# Autodesk Inventor assembly: Assembly_components
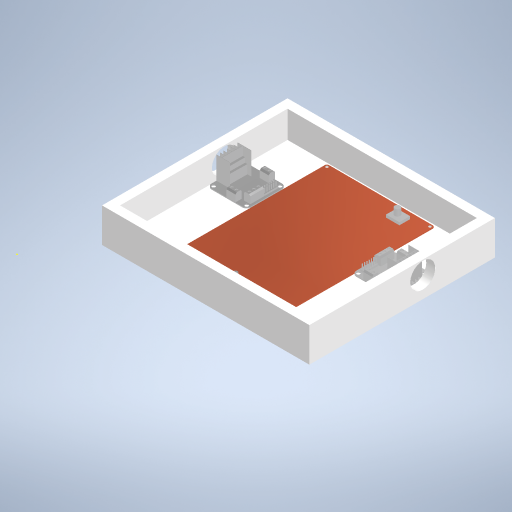
[picture p0: Inventor's stored thumbnail of the model, 512x512]
Saved by Autodesk Inventor 2023 (Build 270158000, 158)
## iProperties
Created: 2023-03-21
Part Number: Assembly_components
Document SubType Name: Assembly
Designer: 55119
Author: 55119
## Documents named in this file (5)
- C:\Users\55119\Documents\GitHub\tectonics\src\3d_models\Case\Assembly_components.iam
- C:\Users\55119\Documents\GitHub\tectonics\src\3d_models\Case\PCB.ipt
- C:\Users\55119\Documents\GitHub\tectonics\src\3d_models\Case\Ponte_H.ipt
- C:\Users\55119\Downloads\Case.ipt
- C:\Users\55119\Documents\GitHub\tectonics\src\3d_models\Case\Case_3d_model.ipt
## Components (5 placed, 4 different names)
1. PCB:1 — Mate:1, Mate:4, Mate:5
2. Ponte_H:1 — Mate:2, Mate:5
3. Case:1 — Mate:1, Mate:2, Mate:3
4. Ponte_H:2 — Mate:3, Mate:4
5. Case_3d_model:1
## Relationships (5: Mate 5)
- Mate:1: PCB:1 ↔ Case:1
- Mate:2: Ponte_H:1 ↔ Case:1
- Mate:3: Case:1 ↔ Ponte_H:2
- Mate:4: PCB:1 ↔ Ponte_H:2
- Mate:5: PCB:1 ↔ Ponte_H:1
